# Autodesk Inventor assembly: tread roller assembly
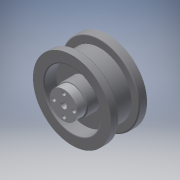
[picture p0: Inventor's stored thumbnail of the model, 180x180]
Saved by Autodesk Inventor 2019 (Build 230136000, 136)
## iProperties
Created: 2019-04-25
Part Number: tread roller assembly
Document SubType Name: Assembly
Designer: User
Author: User
## Documents named in this file (3)
- C:\Robotics\CAD\2019-20_CAD\offseason\random ideas\mecanum tracks\tread roller assembly.iam
- C:\Robotics\CAD\COTSParts\Tetrix\Tetrix Hub - axle.ipt
- C:\Robotics\CAD\COTSParts\Tetrix\Tetrix tread idler wheel.ipt
## Components (3 placed, 2 different names)
1. Tetrix Hub - axle:1 — Mate:1, Mate:2, Mate:3, Mate:6
2. Tetrix Hub - axle:2 — Mate:4, Mate:5, Mate:6
3. Tetrix tread idler wheel:1 — Mate:1, Mate:2, Mate:3, Mate:4, Mate:5
## Relationships (6: Mate 6)
- Mate:1: Tetrix Hub - axle:1 ↔ Tetrix tread idler wheel:1
- Mate:2: Tetrix Hub - axle:1 ↔ Tetrix tread idler wheel:1
- Mate:3: Tetrix Hub - axle:1 ↔ Tetrix tread idler wheel:1
- Mate:4: Tetrix Hub - axle:2 ↔ Tetrix tread idler wheel:1
- Mate:5: Tetrix Hub - axle:2 ↔ Tetrix tread idler wheel:1
- Mate:6: Tetrix Hub - axle:1 ↔ Tetrix Hub - axle:2
